# Autodesk Inventor assembly: EL2-GB-200
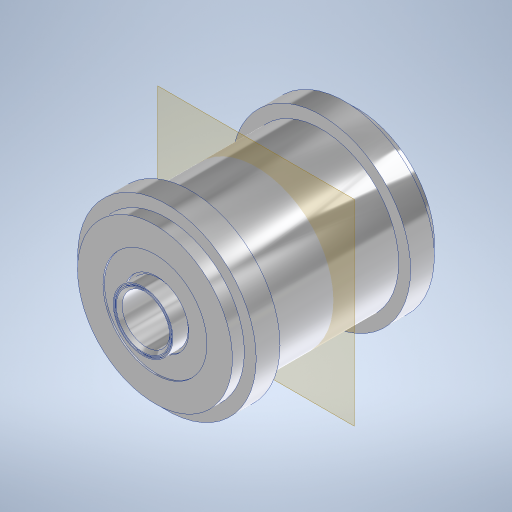
[picture p0: Inventor's stored thumbnail of the model, 512x512]
Saved by Autodesk Inventor 2023.4 (Build 274418000, 418)
## iProperties
Created: 2025-01-11
Part Number: EL2-GB-200
Document SubType Name: Assembly
Designer: mavericks
Author: mavericks
## Documents named in this file (3)
- C:\Users\jmcintyr\Documents\GitHub\2025-ReefScape---CAD\Elevator\EL2-GB\EL2-GB-200.iam
- C:\Users\jmcintyr\Documents\GitHub\2025-ReefScape---CAD\Elevator\EL2\EL2-007.ipt
- C:\Users\jmcintyr\Documents\GitHub\2025-ReefScape---CAD\COMMON PARTS\BEARINGS\.25_Bearing_ext_race.ipt
## Components (3 placed, 2 different names)
1. EL2-007:1 — Mate:1, Mate:2, Mate:3, Mate:4
2. .25_Bearing_ext_race:1 — Mate:3, Mate:4
3. .25_Bearing_ext_race:2 — Mate:1, Mate:2
## Relationships (4: Mate 4)
- Mate:1: EL2-007:1 ↔ .25_Bearing_ext_race:2
- Mate:2: EL2-007:1 ↔ .25_Bearing_ext_race:2
- Mate:3: EL2-007:1 ↔ .25_Bearing_ext_race:1
- Mate:4: EL2-007:1 ↔ .25_Bearing_ext_race:1
